# Autodesk Inventor assembly: Montagem da garra festo
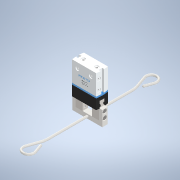
[picture p0: Inventor's stored thumbnail of the model, 180x180]
Saved by Autodesk Inventor 2021 (Build 250183000, 183)
## iProperties
Created: 2013-05-28
Part Number: Montagem da garra festo
Document SubType Name: Assembly
Designer: Kling
Sending System: SolidWorks 2014
Last Author: Marcio Amorim
Last Saved: 2014-05-08
Author: Kling
## Documents named in this file (6)
- C:\Users\rkhaa\OneDrive\Maskinteknik\5. semester\EiT\Inventor\Montagem da garra festo.iam
- C:\Users\rkhaa\OneDrive\Maskinteknik\5. semester\EiT\Inventor\corpo da garra.ipt
- C:\Users\rkhaa\OneDrive\Maskinteknik\5. semester\EiT\Inventor\garra do cilindro.ipt
- C:\Users\rkhaa\OneDrive\Maskinteknik\5. semester\EiT\Inventor\Gripper arm.ipt
- C:\Users\rkhaa\OneDrive\Maskinteknik\5. semester\EiT\Inventor\Rebar type 1.ipt
- C:\Users\rkhaa\Documents\Inventor\Content Center Files\R2021\en-US\ISO 4762(2)\ISO 4762 - M4 x 6ISO.ipt
## Components (10 placed, 5 different names)
1. corpo da garra:1 — Mate:2, Mate:3, Mate:4, Mate:5, Flush:1
2. garra do cilindro:2 — Mate:1, Mate:2, Mate:3, Mate:6, Mate:7, Mate:11
3. garra do cilindro:3 — Mate:4, Mate:5, Mate:6, Flush:1, Mate:8, Mate:9, Mate:10
4. Gripper arm:1 — Mate:1, Mate:7, Mate:11, Mate:12, Mate:13, Insert:1, Insert:2
5. Gripper arm:2 — Mate:8, Mate:9, Mate:10, Insert:3, Insert:4
6. Rebar type 1:1 — Mate:12, Mate:13
7. ISO 4762 M4 x 6:1 — Insert:1
8. ISO 4762 M4 x 6:2 — Insert:2
9. ISO 4762 M4 x 6:3 — Insert:3
10. ISO 4762 M4 x 6:4 — Insert:4
## Relationships (18: Mate 13, Insert 4, Flush 1)
- Mate:1: garra do cilindro:2 ↔ Gripper arm:1
- Mate:2: corpo da garra:1 ↔ garra do cilindro:2
- Mate:3: corpo da garra:1 ↔ garra do cilindro:2
- Mate:4: corpo da garra:1 ↔ garra do cilindro:3
- Mate:5: corpo da garra:1 ↔ garra do cilindro:3
- Mate:6: garra do cilindro:2 ↔ garra do cilindro:3
- Flush:1 (-2.5 mm): corpo da garra:1 ↔ garra do cilindro:3
- Mate:7: garra do cilindro:2 ↔ Gripper arm:1
- Mate:8: garra do cilindro:3 ↔ Gripper arm:2
- Mate:9: garra do cilindro:3 ↔ Gripper arm:2
- Mate:10: garra do cilindro:3 ↔ Gripper arm:2
- Mate:11: garra do cilindro:2 ↔ Gripper arm:1
- Mate:12: Gripper arm:1 ↔ Rebar type 1:1
- Mate:13 (110 mm): Gripper arm:1 ↔ Rebar type 1:1
- Insert:1: Gripper arm:1 ↔ ISO 4762 M4 x 6:1
- Insert:2: Gripper arm:1 ↔ ISO 4762 M4 x 6:2
- Insert:3: Gripper arm:2 ↔ ISO 4762 M4 x 6:3
- Insert:4: Gripper arm:2 ↔ ISO 4762 M4 x 6:4
